# Autodesk Inventor assembly: model_ris
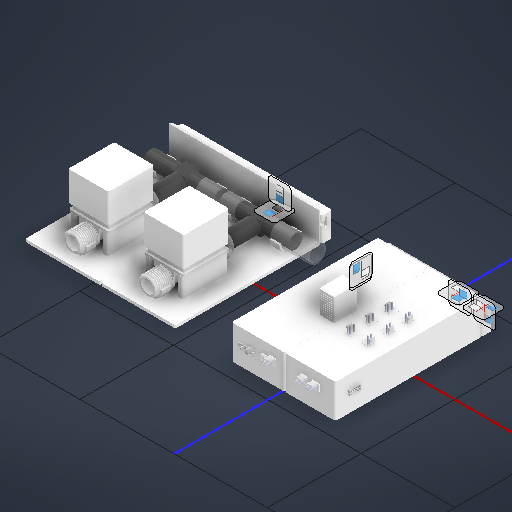
[picture p0: Inventor's stored thumbnail of the model, 512x512]
Saved by Autodesk Inventor 2025.2 (Build 292293000, 293)
## iProperties
Created: 2025-09-05
Part Number: model_ris
Document SubType Name: Assembly
Designer: sam
Author: sam
## Documents named in this file (6)
- G:\projects\primary\regulated-irrigation-system\model\asm\model_ris.iam
- G:\projects\primary\regulated-irrigation-system\model\asm\module-command\module_command.iam
- G:\projects\primary\regulated-irrigation-system\model\asm\module-switch\module_switch.iam
- G:\projects\primary\regulated-irrigation-system\model\asm\module-slot\module-slot.ipt
- G:\projects\primary\regulated-irrigation-system\model\asm\module-valve\module_valve.iam
- G:\projects\primary\regulated-irrigation-system\model\asm\module-slot\module-slot_v2.ipt
## Components (6 placed, 5 different names)
1. module_command:1 [sub-assembly] — Mate:1, Mate:2, Mate:3, Mate:4
2. module_switch:1 [sub-assembly] — Mate:4, Mate:5, Mate:6
3. module-slot:1 — Mate:1, Mate:2, Mate:3, Mate:5, Mate:6, Mate:7, Flush:1, Flush:2
4. module_valve:1 [sub-assembly] — Mate:8, Mate:9, Mate:10, Mate:11
5. module_valve:2 [sub-assembly] — Mate:11, Mate:12, Mate:13
6. module-slot_v2:1 — Mate:7, Mate:8, Mate:9, Mate:10, Flush:1, Flush:2, Mate:12, Mate:13
## Relationships (15: Mate 13, Flush 2)
- Mate:1: module_command:1 ↔ module-slot:1
- Mate:2 (0.2 mm): module_command:1 ↔ module-slot:1
- Mate:3 (0.2 mm): module_command:1 ↔ module-slot:1
- Mate:4: module_command:1 ↔ module_switch:1
- Mate:5 (0.2 mm): module_switch:1 ↔ module-slot:1
- Mate:6 (0.2 mm): module_switch:1 ↔ module-slot:1
- Mate:7 (60 mm): module-slot:1 ↔ module-slot_v2:1
- Mate:8: module_valve:1 ↔ module-slot_v2:1
- Mate:9 (0.2 mm): module_valve:1 ↔ module-slot_v2:1
- Mate:10 (0.2 mm): module_valve:1 ↔ module-slot_v2:1
- Flush:1: module-slot:1 ↔ module-slot_v2:1
- Flush:2: module-slot:1 ↔ module-slot_v2:1
- Mate:11: module_valve:1 ↔ module_valve:2
- Mate:12 (0.2 mm): module_valve:2 ↔ module-slot_v2:1
- Mate:13 (0.2 mm): module_valve:2 ↔ module-slot_v2:1
